# Autodesk Inventor assembly: HalfElevatpr
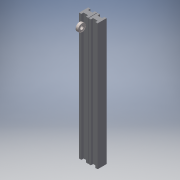
[picture p0: Inventor's stored thumbnail of the model, 180x180]
Saved by Autodesk Inventor 2019 (Build 230136000, 136)
## iProperties
Created: 2019-09-28
Part Number: HalfElevatpr
Document SubType Name: Assembly
Designer: james
Author: james
## Documents named in this file (3)
- F:\JimsDesign\Jims2020FTC\HalfElevatpr.iam
- F:\JimsDesign\Jims2020FTC\LeftSideElevator.ipt
- F:\JimsDesign\Library\AndyMark\am-0516 0.375'' id bearing, shielded (R6ZZ).ipt
## Components (3 placed, 2 different names)
1. LeftSideElevator:1 — Mate:1, Mate:2, Flush:1, Flush:2
2. am-0516 0.375'' id bearing, shielded (R6ZZ):1 — Mate:1
3. LeftSideElevator:2 — Mate:2, Flush:1, Flush:2
## Relationships (4: Mate 2, Flush 2)
- Mate:1: LeftSideElevator:1 ↔ am-0516 0.375'' id bearing, shielded (R6ZZ):1
- Mate:2 (1.27 mm): LeftSideElevator:1 ↔ LeftSideElevator:2
- Flush:1: LeftSideElevator:1 ↔ LeftSideElevator:2
- Flush:2: LeftSideElevator:1 ↔ LeftSideElevator:2
